# Autodesk Inventor assembly: гроб для задницы цел нормис
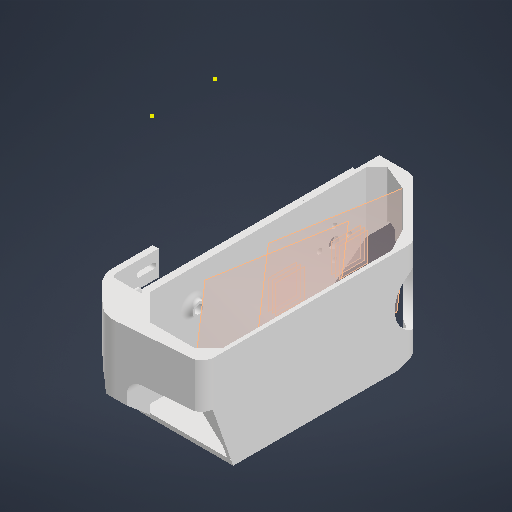
[picture p0: Inventor's stored thumbnail of the model, 512x512]
Saved by Autodesk Inventor 2025 (Build 290162000, 162)
## iProperties
Created: 2024-09-20
Part Number: гроб для задницы цел нормис
Document SubType Name: Assembly
Designer: GameHD
Author: GameHD
## Documents named in this file (3)
- C:\Users\GameHD\Desktop\что-то нужное\Phantom16950\гроб для задницы цел нормис.iam
- C:\Users\GameHD\Desktop\что-то нужное\Phantom16950\гроб для задницы нормис 2Ч.ipt
- C:\Users\GameHD\Desktop\что-то нужное\Phantom16950\гроб для задницы нормис.ipt
## Components (2 placed, 2 different names)
1. гроб для задницы нормис 2Ч:1 — Совмещение:1, Заподлицо:1, Заподлицо:2
2. гроб для задницы нормис:1 — Совмещение:1, Заподлицо:1, Заподлицо:2
## Relationships (3: Flush 2, Mate 1)
- Совмещение:1 [Mate]: гроб для задницы нормис 2Ч:1 ↔ гроб для задницы нормис:1
- Заподлицо:1 [Flush]: гроб для задницы нормис 2Ч:1 ↔ гроб для задницы нормис:1
- Заподлицо:2 [Flush]: гроб для задницы нормис 2Ч:1 ↔ гроб для задницы нормис:1
